# Autodesk Inventor assembly: frame assembly 8
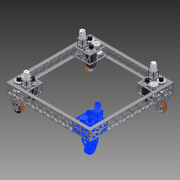
[picture p0: Inventor's stored thumbnail of the model, 180x180]
Saved by Autodesk Inventor 2012 (Build 160160000, 160)
## iProperties
Created: 2013-08-08
Part Number: frame assembly 8
Document SubType Name: Assembly
Designer: Bryce
Author: Bryce
## Documents named in this file (3)
- C:\Users\Bryce\Dropbox\Inventor Design Project Files\Independent Swerves\Inventor 2012\frame assembly 8.iam
- C:\Users\Bryce\Dropbox\Inventor Design Project Files\Independent Swerves\Inventor 2012\FULL SWERVE DRIVE ASSEMBLY!  4!.iam
- C:\Users\Bryce\Dropbox\Inventor Design Project Files\Independent Swerves\Inventor 2012\big U channel 3.25in.ipt
## Components (8 placed, 2 different names)
1. FULL SWERVE DRIVE ASSEMBLY!  4!:1 [sub-assembly] — Mate:1, Mate:2, Mate:4, Mate:5
2. FULL SWERVE DRIVE ASSEMBLY!  4!:2 [sub-assembly] — Mate:19, Mate:20, Mate:21
3. FULL SWERVE DRIVE ASSEMBLY!  4!:3 [sub-assembly] — Mate:7, Mate:8, Mate:9, Mate:10
4. FULL SWERVE DRIVE ASSEMBLY!  4!:4 [sub-assembly] — Mate:13, Mate:14, Mate:17, Mate:18
5. big U channel 3.25in:1 — Mate:1, Mate:2, Mate:3, Mate:6, Mate:19, Mate:20
6. big U channel 3.25in:2 — Mate:3, Mate:4, Mate:5, Mate:6, Mate:7, Mate:8, Mate:11, Mate:12
7. big U channel 3.25in:3 — Mate:9, Mate:10, Mate:11, Mate:12, Mate:13, Mate:14, Mate:15, Mate:16
8. big U channel 3.25in:4 — Mate:15, Mate:16, Mate:17, Mate:18, Mate:21
## Relationships (21: Mate 21)
- Mate:1: FULL SWERVE DRIVE ASSEMBLY!  4!:1 ↔ big U channel 3.25in:1
- Mate:2: FULL SWERVE DRIVE ASSEMBLY!  4!:1 ↔ big U channel 3.25in:1
- Mate:3: big U channel 3.25in:1 ↔ big U channel 3.25in:2
- Mate:4: FULL SWERVE DRIVE ASSEMBLY!  4!:1 ↔ big U channel 3.25in:2
- Mate:5: FULL SWERVE DRIVE ASSEMBLY!  4!:1 ↔ big U channel 3.25in:2
- Mate:6: big U channel 3.25in:1 ↔ big U channel 3.25in:2
- Mate:7: FULL SWERVE DRIVE ASSEMBLY!  4!:3 ↔ big U channel 3.25in:2
- Mate:8: FULL SWERVE DRIVE ASSEMBLY!  4!:3 ↔ big U channel 3.25in:2
- Mate:9: FULL SWERVE DRIVE ASSEMBLY!  4!:3 ↔ big U channel 3.25in:3
- Mate:10: FULL SWERVE DRIVE ASSEMBLY!  4!:3 ↔ big U channel 3.25in:3
- Mate:11: big U channel 3.25in:2 ↔ big U channel 3.25in:3
- Mate:12: big U channel 3.25in:2 ↔ big U channel 3.25in:3
- Mate:13: FULL SWERVE DRIVE ASSEMBLY!  4!:4 ↔ big U channel 3.25in:3
- Mate:14: FULL SWERVE DRIVE ASSEMBLY!  4!:4 ↔ big U channel 3.25in:3
- Mate:15: big U channel 3.25in:3 ↔ big U channel 3.25in:4
- Mate:16: big U channel 3.25in:3 ↔ big U channel 3.25in:4
- Mate:17: FULL SWERVE DRIVE ASSEMBLY!  4!:4 ↔ big U channel 3.25in:4
- Mate:18: FULL SWERVE DRIVE ASSEMBLY!  4!:4 ↔ big U channel 3.25in:4
- Mate:19: FULL SWERVE DRIVE ASSEMBLY!  4!:2 ↔ big U channel 3.25in:1
- Mate:20: FULL SWERVE DRIVE ASSEMBLY!  4!:2 ↔ big U channel 3.25in:1
- Mate:21: FULL SWERVE DRIVE ASSEMBLY!  4!:2 ↔ big U channel 3.25in:4
